# Autodesk Inventor assembly: mount_v2
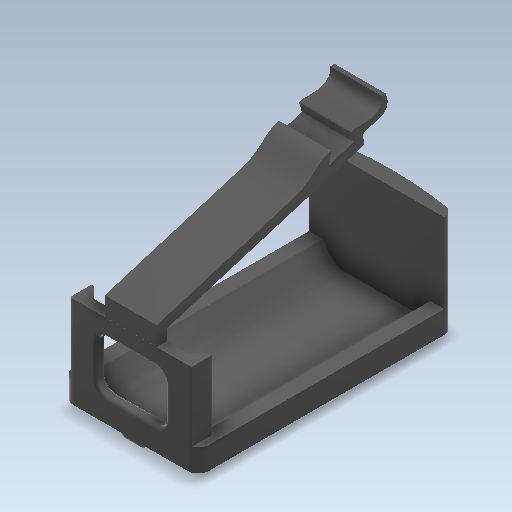
[picture p0: Inventor's stored thumbnail of the model, 512x512]
Saved by Autodesk Inventor 2020 (Build 240168000, 168)
## iProperties
Created: 2024-02-13
Part Number: mount_v2
Document SubType Name: Assembly
Designer: 4s
Author: 4s
## Documents named in this file (3)
- C:\Users\4s\Documents\Inventor models\Asterisk\robot_v2\Bat_mount\mount_v2.iam
- C:\Users\4s\Documents\Inventor models\Asterisk\robot_v2\Bat_mount\bat_mount003.ipt
- C:\Users\4s\Documents\Inventor models\Asterisk\robot_v2\Bat_mount\bat_lock03.ipt
## Components (2 placed, 2 different names)
1. bat_mount003:1 — Заподлицо:1, Совмещение:1, Заподлицо:2, Совмещение:2, Совмещение:3, Заподлицо:3, Заподлицо:4, Заподлицо:5, Совмещение:4
2. bat_lock03:1 — Совмещение:3, Заподлицо:3, Заподлицо:4, Заподлицо:5, Совмещение:4
## Relationships (9: Flush 5, Mate 4)
- Заподлицо:1 [Flush]: bat_mount003:1
- Совмещение:1 [Mate]: bat_mount003:1
- Заподлицо:2 [Flush]: bat_mount003:1
- Совмещение:2 [Mate]: bat_mount003:1
- Совмещение:3 [Mate] (-3.5 mm): bat_mount003:1 ↔ bat_lock03:1
- Заподлицо:3 [Flush]: bat_mount003:1 ↔ bat_lock03:1
- Заподлицо:4 [Flush] (10 mm): bat_mount003:1 ↔ bat_lock03:1
- Заподлицо:5 [Flush] (0.05 mm): bat_mount003:1 ↔ bat_lock03:1
- Совмещение:4 [Mate] (-3.5 mm): bat_mount003:1 ↔ bat_lock03:1
